# Autodesk Inventor assembly: GFRP_T2_07
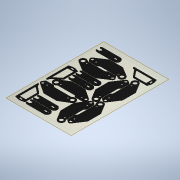
[picture p0: Inventor's stored thumbnail of the model, 180x180]
Saved by Autodesk Inventor 2020 (Build 240168000, 168)
## iProperties
Created: 2021-08-27
Part Number: GFRP_T2_07
Document SubType Name: Assembly
Designer: Masato
Author: Masato
## Documents named in this file (5)
- C:\Users\naoki\Documents\Inventor\CitBrains\git_clone\SUSTAINA_ver1_0\A_T2_175\SUSTAINA-OP\Cam\GFRP_T2_07.iam
- C:\Users\naoki\Documents\Inventor\CitBrains\git_clone\SUSTAINA_ver1_0\A_T2_175\SUSTAINA-OP\Cam\DisposableBoard.ipt
- C:\Users\naoki\Documents\Inventor\CitBrains\git_clone\SUSTAINA_ver1_0\A_T2_175\SUSTAINA-OP\LowerBody\Link\FrontLink_frame.ipt
- C:\Users\naoki\Documents\Inventor\CitBrains\git_clone\SUSTAINA_ver1_0\A_T2_175\SUSTAINA-OP\UpperBody\Arm\UpperArm_side_frame.ipt
- C:\Users\naoki\Documents\Inventor\CitBrains\git_clone\SUSTAINA_ver1_0\A_T2_175\SUSTAINA-OP\UpperBody\Arm\ForeArm_inside_frame.ipt
## Components (17 placed, 4 different names)
1. DisposableBoard:1 — メイト:2, メイト:1, フラッシュ:1, フラッシュ:2, メイト:9, 正接:5, メイト:18, メイト:19, 角度:3, 角度:4, メイト:25, メイト:26, メイト:31, メイト:32, メイト:33, 角度:6, 正接:20, メイト:41, 角度:8, 正接:23, メイト:43, フラッシュ:4, メイト:45, メイト:46, フラッシュ:5, フラッシュ:6, メイト:47, メイト:48, フラッシュ:7, 角度:9, メイト:51, フラッシュ:8, 角度:10, 正接:31, メイト:52
2. FrontLink_frame:2 — メイト:9, 正接:5, メイト:17, 正接:17, 正接:22, 正接:28, 正接:32
3. FrontLink_frame:6 — メイト:16, メイト:18, 正接:12, 正接:13, 正接:22
4. FrontLink_frame:7 — メイト:16, メイト:19, 角度:4, 正接:13, 正接:24
5. FrontLink_frame:8 — メイト:17, 角度:3, メイト:31, 正接:12, 正接:17
6. FrontLink_frame:9 — メイト:25, 正接:27, 角度:9, 正接:28, 正接:29, 正接:31
7. FrontLink_frame:10 — メイト:26, 正接:29, メイト:50, 正接:30, 角度:10, 正接:32
8. UpperArm_side_frame:3 — メイト:41, 角度:8, 正接:24, フラッシュ:4
9. FrontLink_frame:14 — メイト:32, 角度:6, 角度:7, メイト:38, 正接:19, メイト:42
10. FrontLink_frame:15 — メイト:33, 角度:7, メイト:38, 正接:19, 正接:20, メイト:54
11. ForeArm_inside_frame:2 — メイト:42, 正接:23, メイト:43
12. ForeArm_inside_frame:3 — メイト:45, メイト:50, 正接:33, メイト:53
13. UpperArm_side_frame:4 — メイト:46, フラッシュ:5, フラッシュ:6, 正接:25, 正接:26, 正接:27
14. ForeArm_inside_frame:4 — メイト:48, 正接:26, メイト:49
15. ForeArm_inside_frame:5 — メイト:47, フラッシュ:7, 正接:25, メイト:49
16. UpperArm_side_frame:5 — メイト:51, 正接:30, フラッシュ:8, 正接:33, 正接:34
17. ForeArm_inside_frame:6 — メイト:52, メイト:53, メイト:54, 正接:34
## Relationships (59: Mate 26, Tangent 19, Flush 7, Angle 7)
- メイト:2 [Mate]: DisposableBoard:1
- メイト:1 [Mate]: DisposableBoard:1
- フラッシュ:1 [Flush]: DisposableBoard:1
- フラッシュ:2 [Flush]: DisposableBoard:1
- メイト:9 [Mate]: DisposableBoard:1 ↔ FrontLink_frame:2
- 正接:5 [Tangent] (2.5 mm): DisposableBoard:1 ↔ FrontLink_frame:2
- メイト:16 [Mate] (2.5 mm): FrontLink_frame:6 ↔ FrontLink_frame:7
- メイト:17 [Mate] (2.5 mm): FrontLink_frame:2 ↔ FrontLink_frame:8
- メイト:18 [Mate]: DisposableBoard:1 ↔ FrontLink_frame:6
- メイト:19 [Mate]: DisposableBoard:1 ↔ FrontLink_frame:7
- 角度:3 [Angle] (0 deg): DisposableBoard:1 ↔ FrontLink_frame:8
- 角度:4 [Angle] (0 deg): DisposableBoard:1 ↔ FrontLink_frame:7
- メイト:25 [Mate]: DisposableBoard:1 ↔ FrontLink_frame:9
- メイト:26 [Mate]: DisposableBoard:1 ↔ FrontLink_frame:10
- メイト:31 [Mate]: DisposableBoard:1 ↔ FrontLink_frame:8
- 正接:12 [Tangent] (2.5 mm): FrontLink_frame:6 ↔ FrontLink_frame:8
- 正接:13 [Tangent] (3 mm): FrontLink_frame:6 ↔ FrontLink_frame:7
- 正接:17 [Tangent] (3 mm): FrontLink_frame:2 ↔ FrontLink_frame:8
- メイト:32 [Mate]: DisposableBoard:1 ↔ FrontLink_frame:14
- メイト:33 [Mate]: DisposableBoard:1 ↔ FrontLink_frame:15
- 角度:6 [Angle] (0 deg): DisposableBoard:1 ↔ FrontLink_frame:14
- 角度:7 [Angle] (0 deg): FrontLink_frame:14 ↔ FrontLink_frame:15
- メイト:38 [Mate] (2.5 mm): FrontLink_frame:14 ↔ FrontLink_frame:15
- 正接:19 [Tangent] (3 mm): FrontLink_frame:14 ↔ FrontLink_frame:15
- 正接:20 [Tangent] (2 mm): DisposableBoard:1 ↔ FrontLink_frame:15
- 正接:22 [Tangent] (2.5 mm): FrontLink_frame:2 ↔ FrontLink_frame:6
- メイト:41 [Mate]: DisposableBoard:1 ↔ UpperArm_side_frame:3
- 角度:8 [Angle] (0 deg): DisposableBoard:1 ↔ UpperArm_side_frame:3
- メイト:42 [Mate] (2.5 mm): FrontLink_frame:14 ↔ ForeArm_inside_frame:2
- 正接:23 [Tangent] (2 mm): DisposableBoard:1 ↔ ForeArm_inside_frame:2
- メイト:43 [Mate]: DisposableBoard:1 ↔ ForeArm_inside_frame:2
- 正接:24 [Tangent] (2.5 mm): FrontLink_frame:7 ↔ UpperArm_side_frame:3
- フラッシュ:4 [Flush] (4 mm): DisposableBoard:1 ↔ UpperArm_side_frame:3
- メイト:45 [Mate]: DisposableBoard:1 ↔ ForeArm_inside_frame:3
- メイト:46 [Mate]: DisposableBoard:1 ↔ UpperArm_side_frame:4
- フラッシュ:5 [Flush] (2 mm): DisposableBoard:1 ↔ UpperArm_side_frame:4
- フラッシュ:6 [Flush] (2 mm): DisposableBoard:1 ↔ UpperArm_side_frame:4
- メイト:47 [Mate]: DisposableBoard:1 ↔ ForeArm_inside_frame:5
- メイト:48 [Mate]: DisposableBoard:1 ↔ ForeArm_inside_frame:4
- フラッシュ:7 [Flush] (2 mm): DisposableBoard:1 ↔ ForeArm_inside_frame:5
- 正接:25 [Tangent] (2.5 mm): UpperArm_side_frame:4 ↔ ForeArm_inside_frame:5
- 正接:26 [Tangent] (2.5 mm): UpperArm_side_frame:4 ↔ ForeArm_inside_frame:4
- メイト:49 [Mate] (2.5 mm): ForeArm_inside_frame:4 ↔ ForeArm_inside_frame:5
- 正接:27 [Tangent] (2.5 mm): FrontLink_frame:9 ↔ UpperArm_side_frame:4
- 角度:9 [Angle] (0 deg): DisposableBoard:1 ↔ FrontLink_frame:9
- 正接:28 [Tangent] (2.5 mm): FrontLink_frame:2 ↔ FrontLink_frame:9
- 正接:29 [Tangent] (2.5 mm): FrontLink_frame:9 ↔ FrontLink_frame:10
- メイト:50 [Mate] (2.5 mm): FrontLink_frame:10 ↔ ForeArm_inside_frame:3
- メイト:51 [Mate]: DisposableBoard:1 ↔ UpperArm_side_frame:5
- 正接:30 [Tangent] (2.5 mm): FrontLink_frame:10 ↔ UpperArm_side_frame:5
- フラッシュ:8 [Flush] (2 mm): DisposableBoard:1 ↔ UpperArm_side_frame:5
- 角度:10 [Angle] (0 deg): DisposableBoard:1 ↔ FrontLink_frame:10
- 正接:31 [Tangent] (2 mm): DisposableBoard:1 ↔ FrontLink_frame:9
- 正接:32 [Tangent] (2.5 mm): FrontLink_frame:2 ↔ FrontLink_frame:10
- 正接:33 [Tangent] (2.5 mm): ForeArm_inside_frame:3 ↔ UpperArm_side_frame:5
- メイト:52 [Mate]: DisposableBoard:1 ↔ ForeArm_inside_frame:6
- メイト:53 [Mate] (2.5 mm): ForeArm_inside_frame:3 ↔ ForeArm_inside_frame:6
- メイト:54 [Mate] (2.5 mm): FrontLink_frame:15 ↔ ForeArm_inside_frame:6
- 正接:34 [Tangent] (2.5 mm): UpperArm_side_frame:5 ↔ ForeArm_inside_frame:6
